# Autodesk Inventor assembly: КВ33.044.200 - Каретка оси Х
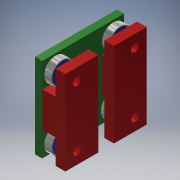
[picture p0: Inventor's stored thumbnail of the model, 180x180]
Saved by Autodesk Inventor 2019 (Build 230136000, 136)
## iProperties
Created: 2019-07-16
Part Number: КВ33.044.200 - Каретка оси Х
Material: Типовые
Document SubType Name: Assembly
Designer: Петров Иван
Author: Петров Иван
## Documents named in this file (4)
- C:\Users\user\Documents\Kvantoriada2019\optimal_gripper\hardware\КВ33.044.200 - Каретка оси Х.iam
- C:\Users\user\Documents\Kvantoriada2019\optimal_gripper\hardware\КВ33.044.201 - Щека каретки.ipt
- C:\Users\user\Documents\Kvantoriada2019\optimal_gripper\hardware\Стандартные изделия\Подшипник 626Z.ipt
- C:\Users\user\Documents\Kvantoriada2019\optimal_gripper\hardware\КВ33.044.202 - Фиксатор каретки.ipt
## Components (7 placed, 3 different names)
1. КВ33.044.201 - Щека каретки:1 — Совмещение:1, Совмещение:2, Совмещение:3, Совмещение:4, Совмещение:5, Совмещение:6, Совмещение:7, Совмещение:8, Совмещение:10, Совмещение:14
2. Подшипник 626Z:1 — Совмещение:1, Совмещение:2, Совмещение:11
3. Подшипник 626Z:2 — Совмещение:3, Совмещение:6, Совмещение:12
4. Подшипник 626Z:3 — Совмещение:5, Совмещение:8, Совмещение:13
5. Подшипник 626Z:4 — Совмещение:4, Совмещение:7, Совмещение:9
6. КВ33.044.202 - Фиксатор каретки:1 — Совмещение:9, Совмещение:10, Совмещение:11
7. КВ33.044.202 - Фиксатор каретки:2 — Совмещение:12, Совмещение:13, Совмещение:14
## Relationships (14: Mate 14)
- Совмещение:1 [Mate]: КВ33.044.201 - Щека каретки:1 ↔ Подшипник 626Z:1
- Совмещение:2 [Mate] (1 mm): КВ33.044.201 - Щека каретки:1 ↔ Подшипник 626Z:1
- Совмещение:3 [Mate]: КВ33.044.201 - Щека каретки:1 ↔ Подшипник 626Z:2
- Совмещение:4 [Mate]: КВ33.044.201 - Щека каретки:1 ↔ Подшипник 626Z:4
- Совмещение:5 [Mate]: КВ33.044.201 - Щека каретки:1 ↔ Подшипник 626Z:3
- Совмещение:6 [Mate] (1 mm): КВ33.044.201 - Щека каретки:1 ↔ Подшипник 626Z:2
- Совмещение:7 [Mate] (1 mm): КВ33.044.201 - Щека каретки:1 ↔ Подшипник 626Z:4
- Совмещение:8 [Mate]: КВ33.044.201 - Щека каретки:1 ↔ Подшипник 626Z:3
- Совмещение:9 [Mate]: Подшипник 626Z:4 ↔ КВ33.044.202 - Фиксатор каретки:1
- Совмещение:10 [Mate]: КВ33.044.201 - Щека каретки:1 ↔ КВ33.044.202 - Фиксатор каретки:1
- Совмещение:11 [Mate]: Подшипник 626Z:1 ↔ КВ33.044.202 - Фиксатор каретки:1
- Совмещение:12 [Mate]: Подшипник 626Z:2 ↔ КВ33.044.202 - Фиксатор каретки:2
- Совмещение:13 [Mate]: Подшипник 626Z:3 ↔ КВ33.044.202 - Фиксатор каретки:2
- Совмещение:14 [Mate]: КВ33.044.201 - Щека каретки:1 ↔ КВ33.044.202 - Фиксатор каретки:2
